# Autodesk Inventor assembly: Throughput Mockup Assembly
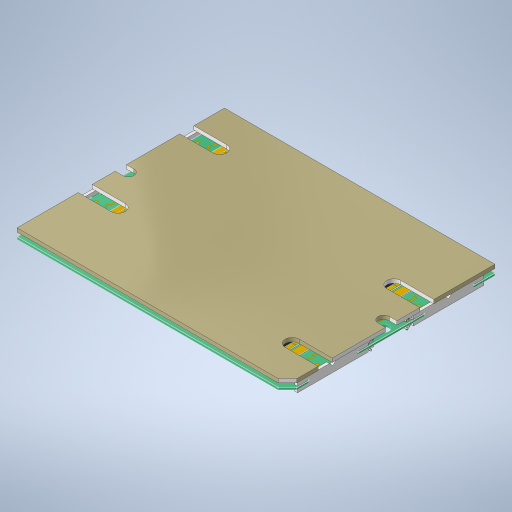
[picture p0: Inventor's stored thumbnail of the model, 512x512]
Saved by Autodesk Inventor 2023 (Build 270158000, 158)
## iProperties
Created: 2022-04-25
Part Number: Throughput Mockup Assembly
Document SubType Name: Assembly
Designer: Caleb
Author: Caleb
## Documents named in this file (7)
- C:\Users\Caleb\Desktop\nebraska-silicon-lab\Hardware\ETL\modules\throughput mockups\Throughput Mockup Assembly.iam
- C:\Users\Caleb\Desktop\nebraska-silicon-lab\Hardware\ETL\modules\throughput mockups\BBM Assembly.iam
- C:\Users\Caleb\Desktop\nebraska-silicon-lab\Hardware\ETL\modules\throughput mockups\Coverplate Film.ipt
- C:\Users\Caleb\Desktop\nebraska-silicon-lab\Hardware\ETL\modules\throughput mockups\Sensor Placement Film.ipt
- C:\Users\Caleb\Desktop\nebraska-silicon-lab\Hardware\ETL\modules\throughput mockups\Baseplate v1.5.ipt
- C:\Users\Caleb\Desktop\nebraska-silicon-lab\Hardware\ETL\modules\throughput mockups\etl_module_pcb_mockup_v3p3p1.ipt
- C:\Users\Caleb\Desktop\nebraska-silicon-lab\Hardware\ETL\modules\tamale v1.4\insert spacer - v1.ipt
## Components (12 placed, 6 different names)
1. BBM Assembly:1 [sub-assembly] — Flush:17, Flush:20, Mate:13, Flush:22
2. BBM Assembly:2 [sub-assembly] — Flush:16, Flush:19, Mate:14, Flush:21, Mate:15, Flush:29, Flush:30
3. BBM Assembly:3 [sub-assembly] — Flush:18, Flush:20, Mate:13, Mate:14, Flush:21
4. BBM Assembly:4 [sub-assembly] — Flush:16, Flush:17, Flush:18, Flush:19, Flush:22, Flush:23, Flush:24, Mate:16, Flush:25, Flush:26
5. Coverplate Film:1 — Mate:12, Mate:16, Flush:25, Flush:26
6. Sensor Placement Film:1 — Mate:15, Flush:23, Flush:24, Mate:17
7. Baseplate v1.5:1 — Mate:12, Flush:27, Flush:28
8. etl_module_pcb_mockup_v3p3p1:1 — Mate:17, Flush:27, Flush:28, Mate:18, Mate:19, Flush:29, Flush:30, Mate:20, Mate:21, Mate:22, Mate:23, Mate:24, Mate:25, Mate:26, Mate:27, Mate:28, Mate:29
9. insert spacer - v1:1 — Mate:18, Mate:19, Mate:29
10. insert spacer - v1:2 — Mate:20, Mate:21, Mate:22
11. insert spacer - v1:3 — Mate:23, Mate:24, Mate:25
12. insert spacer - v1:4 — Mate:26, Mate:27, Mate:28
## Relationships (33: Mate 18, Flush 15)
- Mate:12: Coverplate Film:1 ↔ Baseplate v1.5:1
- Flush:16: BBM Assembly:2 ↔ BBM Assembly:4
- Flush:17: BBM Assembly:1 ↔ BBM Assembly:4
- Flush:18: BBM Assembly:3 ↔ BBM Assembly:4
- Flush:19: BBM Assembly:2 ↔ BBM Assembly:4
- Flush:20: BBM Assembly:1 ↔ BBM Assembly:3
- Mate:13 (0.2 mm): BBM Assembly:1 ↔ BBM Assembly:3
- Mate:14 (0.2 mm): BBM Assembly:2 ↔ BBM Assembly:3
- Flush:21: BBM Assembly:2 ↔ BBM Assembly:3
- Flush:22: BBM Assembly:1 ↔ BBM Assembly:4
- Mate:15: BBM Assembly:2 ↔ Sensor Placement Film:1
- Flush:23: BBM Assembly:4 ↔ Sensor Placement Film:1
- Flush:24: BBM Assembly:4 ↔ Sensor Placement Film:1
- Mate:16: BBM Assembly:4 ↔ Coverplate Film:1
- Flush:25 (0.5 mm): BBM Assembly:4 ↔ Coverplate Film:1
- Flush:26 (0.9 mm): BBM Assembly:4 ↔ Coverplate Film:1
- Mate:17: Sensor Placement Film:1 ↔ etl_module_pcb_mockup_v3p3p1:1
- Flush:27: Baseplate v1.5:1 ↔ etl_module_pcb_mockup_v3p3p1:1
- Flush:28: Baseplate v1.5:1 ↔ etl_module_pcb_mockup_v3p3p1:1
- Mate:18: etl_module_pcb_mockup_v3p3p1:1 ↔ insert spacer - v1:1
- Mate:19: etl_module_pcb_mockup_v3p3p1:1 ↔ insert spacer - v1:1
- Flush:29 (0.75 mm): BBM Assembly:2 ↔ etl_module_pcb_mockup_v3p3p1:1
- Flush:30 (5.45 mm): BBM Assembly:2 ↔ etl_module_pcb_mockup_v3p3p1:1
- Mate:20: etl_module_pcb_mockup_v3p3p1:1 ↔ insert spacer - v1:2
- Mate:21: etl_module_pcb_mockup_v3p3p1:1 ↔ insert spacer - v1:2
- Mate:22: etl_module_pcb_mockup_v3p3p1:1 ↔ insert spacer - v1:2
- Mate:23: etl_module_pcb_mockup_v3p3p1:1 ↔ insert spacer - v1:3
- Mate:24: etl_module_pcb_mockup_v3p3p1:1 ↔ insert spacer - v1:3
- Mate:25: etl_module_pcb_mockup_v3p3p1:1 ↔ insert spacer - v1:3
- Mate:26: etl_module_pcb_mockup_v3p3p1:1 ↔ insert spacer - v1:4
- Mate:27: etl_module_pcb_mockup_v3p3p1:1 ↔ insert spacer - v1:4
- Mate:28: etl_module_pcb_mockup_v3p3p1:1 ↔ insert spacer - v1:4
- Mate:29: etl_module_pcb_mockup_v3p3p1:1 ↔ insert spacer - v1:1
